# Autodesk Inventor assembly: link9_SubAssembly.ipt
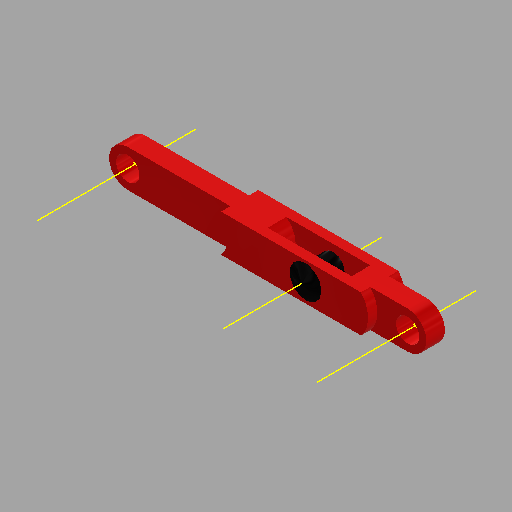
[picture p0: Inventor's stored thumbnail of the model, 512x512]
Saved by Autodesk Inventor 2024.1 (Build 281209000, 209)
## iProperties
Created: 2023-11-11
Part Number: link9_SubAssembly.ipt
Document SubType Name: Assembly
Designer: Camilo
Mass: 0.891544 g
Surface Area: 6.14448 cm^2
Volume: 0.330201 cm^3
Density: 2.7 g/cm^3
Author: Camilo
## Documents named in this file (3)
- D:\Documentos\MEGA\Universidad\2023-2\DinamicaComputacionalDeSistemasMulticuerpo\DinamicaComputacionalSistemasMulticuerpo\Proyecto\CAD\3D\link7_SubAssembly.iam
- D:\Documentos\MEGA\Universidad\2023-2\DinamicaComputacionalDeSistemasMulticuerpo\DinamicaComputacionalSistemasMulticuerpo\Proyecto\CAD\3D\link7.ipt
- D:\Documentos\MEGA\Universidad\2023-2\DinamicaComputacionalDeSistemasMulticuerpo\DinamicaComputacionalSistemasMulticuerpo\Proyecto\CAD\3D\bolt.ipt
## Components (2 placed, 2 different names)
1. link7:1 — Mate:1, Mate:2
2. bolt:1 — Mate:1, Mate:2
## Relationships (2: Mate 2)
- Mate:1: link7:1 ↔ bolt:1
- Mate:2: link7:1 ↔ bolt:1
